# Autodesk Inventor assembly: x_iddler
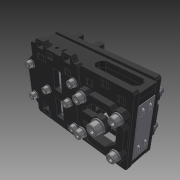
[picture p0: Inventor's stored thumbnail of the model, 180x180]
Saved by Autodesk Inventor 2014 (Build 180170000, 170)
## iProperties
Created: 2014-03-20
Part Number: x_iddler
Document SubType Name: Assembly
Designer: buben
Author: buben
## Documents named in this file (22)
- C:\Users\buben\Documents\GitHub\bacon\inventor files\printer parts\6.5 mm\x_iddler.iam
- C:\Users\buben\Documents\GitHub\bacon\inventor files\printer parts\6.5 mm\x_iddler_bottom.ipt
- C:\Users\buben\Documents\GitHub\bacon\inventor files\printer parts\6.5 mm\x_iddler_belt_bearing_mount.ipt
- C:\Users\buben\Documents\GitHub\bacon\inventor files\printer parts\6.5 mm\x_motor_smooth_rod_spacer.ipt
- C:\Users\buben\Documents\GitHub\bacon\inventor files\printer parts\6.5 mm\x_iddler_wall_lower.ipt
- C:\Users\buben\Documents\GitHub\bacon\inventor files\printer parts\6.5 mm\x_iddler_wall_upper.ipt
- C:\Users\buben\Documents\GitHub\bacon\inventor files\printer parts\6.5 mm\x_iddler_upper_nut_stop.ipt
- C:\Users\buben\Documents\GitHub\bacon\inventor files\printer parts\6.5 mm\x_motor_middle.ipt
- C:\Users\buben\Documents\GitHub\bacon\inventor files\printer parts\6.5 mm\x_iddler_c_mount.ipt
- C:\Users\buben\Documents\GitHub\bacon\inventor files\printer parts\6.5 mm\x_motor_top.ipt
- C:\Users\buben\Documents\GitHub\bacon\inventor files\printer parts\6.5 mm\x_iddler_right_cap.ipt
- C:\Users\buben\Documents\GitHub\bacon\inventor files\utils\washer_m5.ipt
- C:\Users\buben\Documents\GitHub\bacon\inventor files\utils\washer_m6.ipt
- C:\Users\buben\Documents\Inventor\Content Center Files\R2014\en-US\ISO 4762(2)\ISO 4762 - M6 x 60ISO.ipt
- C:\Users\buben\Documents\GitHub\bacon\inventor files\utils\washer_m8.ipt
- C:\Users\buben\Documents\Inventor\Content Center Files\R2014\en-US\ISO 4762(2)\ISO 4762 - M8 x 65ISO.ipt
- C:\Users\buben\Documents\Inventor\Content Center Files\R2014\en-US\ISO 7040\ISO 7040 - M5.ipt
- C:\Users\buben\Documents\Inventor\Content Center Files\R2014\en-US\ISO 7040\ISO 7040 - M6.ipt
- C:\Users\buben\Documents\Inventor\Content Center Files\R2014\en-US\ISO 7040\ISO 7040 - M8.ipt
- C:\Users\buben\Documents\GitHub\bacon\inventor files\3rd party components\linear_bearing_8\Imported Components\LU8MM\LU8MM.iam
- C:\Users\buben\Documents\Inventor\Content Center Files\R2014\en-US\ISO 4762(2)\ISO 4762 - M5 x 50ISO.ipt
- C:\Users\buben\Documents\GitHub\bacon\inventor files\utils\x_iddler_cap_zip_tie.ipt
## Components (62 placed, 21 different names)
1. x_iddler_bottom:1 — Mate:1, Mate:2, Mate:3, Mate:4, Mate:5, Mate:6, Mate:7, Mate:8, Mate:9, Mate:10, Mate:11, Mate:12, Mate:13, Mate:14, Mate:15, Mate:16, Mate:17, Mate:18, Mate:19, Mate:21, Mate:33, Tangent:1, Mate:41, Mate:42, Mate:43, Mate:44, Mate:45, Mate:46
2. x_iddler_belt_bearing_mount:1 — Mate:4, Mate:5, Mate:6, Mate:67, Mate:68, Mate:69, Mate:70, Mate:76, Mate:77
3. x_motor_smooth_rod_spacer:1 — Mate:7, Mate:10, Mate:12, Mate:22
4. x_motor_smooth_rod_spacer:2 — Mate:8, Mate:9, Mate:11
5. x_iddler_wall_lower:1 — Mate:13, Mate:14, Mate:15, Mate:23, Mate:24, Mate:25, Mate:26, Mate:27, Mate:32, Mate:34
6. x_iddler_wall_upper:1 — Mate:16, Mate:17, Mate:18, Mate:20, Mate:31
7. x_iddler_upper_nut_stop:1 — Mate:19, Mate:20, Mate:21
8. x_motor_middle:1 — Mate:22, Mate:23, Mate:24, Mate:101, Mate:102, Mate:103, Mate:104, Mate:106, Mate:107
9. x_iddler_c_mount:1 — Mate:25, Mate:26, Mate:27, Mate:28, Mate:29, Mate:30
10. x_iddler_belt_bearing_mount:2 — Mate:28, Mate:29, Mate:30, Mate:59, Mate:60, Mate:61, Mate:62, Mate:63, Mate:64, Mate:65, Mate:66, Mate:75, Mate:78
11. x_motor_top:1 — Mate:31, Mate:32, Mate:35, Mate:36, Mate:37, Mate:38, Mate:39, Mate:40, Mate:47, Mate:48, Mate:49, Mate:50, Mate:51, Mate:52, Mate:105
12. x_iddler_right_cap:1 — Mate:33, Mate:34, Tangent:1, Angle:1, Angle:2, Angle:3, Angle:4, Tangent:2, Tangent:3, Tangent:4, Tangent:5
13. CSN 02 1702 B B 5,3:1 — Mate:37, Mate:47, Insert:3
14. CSN 02 1702 B B 5,3:2 — Mate:35, Mate:48, Insert:1
15. CSN 02 1702 B B 5,3:3 — Mate:36, Mate:49, Insert:2
16. CSN 02 1702 B B 5,3:4 — Mate:39, Mate:51, Insert:4
17. CSN 02 1702 B B 5,3:5 — Mate:40, Mate:52, Insert:6
18. CSN 02 1702 B B 5,3:6 — Mate:38, Mate:50, Insert:5
19. CSN 02 1702 B B 5,3:7 — Mate:42, Mate:57, Mate:83
20. CSN 02 1702 B B 5,3:8 — Mate:45, Mate:54, Mate:80
21. CSN 02 1702 B B 5,3:9 — Mate:44, Mate:55, Mate:81
22. CSN 02 1702 B B 5,3:10 — Mate:41, Mate:58, Mate:84
23. CSN 02 1702 B B 5,3:11 — Mate:46, Mate:53, Mate:79
24. CSN 02 1702 B B 5,3:12 — Mate:43, Mate:56, Mate:82
25. ISO 4762 M5 x 50:4 — Insert:4, Mate:57, Mate:88
26. ISO 4762 M5 x 50:2 — Insert:3, Mate:54, Mate:85
27. ISO 4762 M5 x 50:1 — Insert:1, Mate:53, Mate:86
28. ISO 4762 M5 x 50:3 — Insert:2, Mate:55, Mate:87
29. ISO 4762 M5 x 50:5 — Insert:6, Mate:58, Mate:89
30. ISO 4762 M5 x 50:6 — Insert:5, Mate:56, Mate:90
31. ISO 4762 M6 x 60:1 — Insert:8, Mate:73, Mate:96
32. ISO 4762 M6 x 60:4 — Insert:9, Mate:71, Mate:98, Mate:108, Mate:109
33. ISO 4762 M6 x 60:2 — Insert:10, Mate:72, Mate:95, Mate:110, Mate:111
34. ISO 4762 M6 x 60:3 — Insert:7, Mate:74, Mate:97
35. CSN 02 1702 B B 6,4:1 — Mate:59, Mate:65, Insert:7
36. CSN 02 1702 B B 6,4:2 — Mate:61, Mate:66, Insert:9
37. CSN 02 1702 B B 6,4:3 — Mate:60, Mate:64, Insert:8
38. CSN 02 1702 B B 6,4:4 — Mate:62, Mate:63, Insert:10
39. CSN 02 1702 B B 6,4:5 — Mate:68, Mate:72, Mate:92
40. CSN 02 1702 B B 6,4:6 — Mate:67, Mate:71, Mate:91
41. CSN 02 1702 B B 6,4:7 — Mate:69, Mate:73, Mate:94
42. CSN 02 1702 B B 6,4:8 — Mate:70, Mate:74, Mate:93
43. CSN 02 1702 B B 8,4:1 — Mate:76, Mate:77, Mate:99
44. CSN 02 1702 B B 8,4:2 — Mate:75, Mate:78, Insert:11
45. ISO 4762 M8 x 65:1 — Insert:11, Mate:100
46. DIN EN ISO 7040 M5:1 — Mate:83, Mate:88
47. DIN EN ISO 7040 M5:2 — Mate:84, Mate:89
48. DIN EN ISO 7040 M5:3 — Mate:80, Mate:85
49. DIN EN ISO 7040 M5:4 — Mate:81, Mate:87
50. DIN EN ISO 7040 M5:5 — Mate:82, Mate:90
51. DIN EN ISO 7040 M5:6 — Mate:79, Mate:86
52. DIN EN ISO 7040 M6:1 — Mate:92, Mate:95
53. DIN EN ISO 7040 M6:2 — Mate:91, Mate:98
54. DIN EN ISO 7040 M6:3 — Mate:94, Mate:96
55. DIN EN ISO 7040 M6:4 — Mate:93, Mate:97
56. DIN EN ISO 7040 M8:1 — Mate:99, Mate:100
57. LU8MM:1 [sub-assembly] — Mate:101, Mate:102, Mate:107
58. LU8MM:2 [sub-assembly] — Mate:103, Mate:104, Mate:105, Mate:106
59. x_iddler_cap_zip_tie:1 — Mate:109, Angle:3, Tangent:3
60. x_iddler_cap_zip_tie:2 — Mate:108, Angle:4, Tangent:5
61. x_iddler_cap_zip_tie:3 — Mate:110, Angle:2, Tangent:2
62. x_iddler_cap_zip_tie:4 — Mate:111, Angle:1, Tangent:4
## Relationships (131: Mate 111, Insert 11, Tangent 5, Angle 4)
- Mate:1: x_iddler_bottom:1
- Mate:2: x_iddler_bottom:1
- Mate:3: x_iddler_bottom:1
- Mate:4: x_iddler_bottom:1 ↔ x_iddler_belt_bearing_mount:1
- Mate:5: x_iddler_bottom:1 ↔ x_iddler_belt_bearing_mount:1
- Mate:6: x_iddler_bottom:1 ↔ x_iddler_belt_bearing_mount:1
- Mate:7: x_iddler_bottom:1 ↔ x_motor_smooth_rod_spacer:1
- Mate:8: x_iddler_bottom:1 ↔ x_motor_smooth_rod_spacer:2
- Mate:9: x_iddler_bottom:1 ↔ x_motor_smooth_rod_spacer:2
- Mate:10: x_iddler_bottom:1 ↔ x_motor_smooth_rod_spacer:1
- Mate:11: x_iddler_bottom:1 ↔ x_motor_smooth_rod_spacer:2
- Mate:12: x_iddler_bottom:1 ↔ x_motor_smooth_rod_spacer:1
- Mate:13: x_iddler_bottom:1 ↔ x_iddler_wall_lower:1
- Mate:14: x_iddler_bottom:1 ↔ x_iddler_wall_lower:1
- Mate:15: x_iddler_bottom:1 ↔ x_iddler_wall_lower:1
- Mate:16: x_iddler_bottom:1 ↔ x_iddler_wall_upper:1
- Mate:17: x_iddler_bottom:1 ↔ x_iddler_wall_upper:1
- Mate:18: x_iddler_bottom:1 ↔ x_iddler_wall_upper:1
- Mate:19: x_iddler_bottom:1 ↔ x_iddler_upper_nut_stop:1
- Mate:20: x_iddler_wall_upper:1 ↔ x_iddler_upper_nut_stop:1
- Mate:21: x_iddler_bottom:1 ↔ x_iddler_upper_nut_stop:1
- Mate:22: x_motor_smooth_rod_spacer:1 ↔ x_motor_middle:1
- Mate:23: x_iddler_wall_lower:1 ↔ x_motor_middle:1
- Mate:24: x_iddler_wall_lower:1 ↔ x_motor_middle:1
- Mate:25: x_iddler_wall_lower:1 ↔ x_iddler_c_mount:1
- Mate:26: x_iddler_wall_lower:1 ↔ x_iddler_c_mount:1
- Mate:27: x_iddler_wall_lower:1 ↔ x_iddler_c_mount:1
- Mate:28: x_iddler_c_mount:1 ↔ x_iddler_belt_bearing_mount:2
- Mate:29: x_iddler_c_mount:1 ↔ x_iddler_belt_bearing_mount:2
- Mate:30: x_iddler_c_mount:1 ↔ x_iddler_belt_bearing_mount:2
- Mate:31: x_iddler_wall_upper:1 ↔ x_motor_top:1
- Mate:32: x_iddler_wall_lower:1 ↔ x_motor_top:1
- Mate:33: x_iddler_bottom:1 ↔ x_iddler_right_cap:1
- Mate:34: x_iddler_wall_lower:1 ↔ x_iddler_right_cap:1
- Tangent:1: x_iddler_bottom:1 ↔ x_iddler_right_cap:1
- Mate:35: x_motor_top:1 ↔ CSN 02 1702 B B 5,3:2
- Mate:36: x_motor_top:1 ↔ CSN 02 1702 B B 5,3:3
- Mate:37: x_motor_top:1 ↔ CSN 02 1702 B B 5,3:1
- Mate:38: x_motor_top:1 ↔ CSN 02 1702 B B 5,3:6
- Mate:39: x_motor_top:1 ↔ CSN 02 1702 B B 5,3:4
- Mate:40: x_motor_top:1 ↔ CSN 02 1702 B B 5,3:5
- Mate:41: x_iddler_bottom:1 ↔ CSN 02 1702 B B 5,3:10
- Mate:42: x_iddler_bottom:1 ↔ CSN 02 1702 B B 5,3:7
- Mate:43: x_iddler_bottom:1 ↔ CSN 02 1702 B B 5,3:12
- Mate:44: x_iddler_bottom:1 ↔ CSN 02 1702 B B 5,3:9
- Mate:45: x_iddler_bottom:1 ↔ CSN 02 1702 B B 5,3:8
- Mate:46: x_iddler_bottom:1 ↔ CSN 02 1702 B B 5,3:11
- Mate:47: x_motor_top:1 ↔ CSN 02 1702 B B 5,3:1
- Mate:48: x_motor_top:1 ↔ CSN 02 1702 B B 5,3:2
- Mate:49: x_motor_top:1 ↔ CSN 02 1702 B B 5,3:3
- Mate:50: x_motor_top:1 ↔ CSN 02 1702 B B 5,3:6
- Mate:51: x_motor_top:1 ↔ CSN 02 1702 B B 5,3:4
- Mate:52: x_motor_top:1 ↔ CSN 02 1702 B B 5,3:5
- Insert:1: CSN 02 1702 B B 5,3:2 ↔ ISO 4762 M5 x 50:1
- Insert:2: CSN 02 1702 B B 5,3:3 ↔ ISO 4762 M5 x 50:3
- Insert:3: CSN 02 1702 B B 5,3:1 ↔ ISO 4762 M5 x 50:2
- Insert:4: CSN 02 1702 B B 5,3:4 ↔ ISO 4762 M5 x 50:4
- Insert:5: CSN 02 1702 B B 5,3:6 ↔ ISO 4762 M5 x 50:6
- Insert:6: CSN 02 1702 B B 5,3:5 ↔ ISO 4762 M5 x 50:5
- Mate:53: CSN 02 1702 B B 5,3:11 ↔ ISO 4762 M5 x 50:1
- Mate:54: CSN 02 1702 B B 5,3:8 ↔ ISO 4762 M5 x 50:2
- Mate:55: CSN 02 1702 B B 5,3:9 ↔ ISO 4762 M5 x 50:3
- Mate:56: CSN 02 1702 B B 5,3:12 ↔ ISO 4762 M5 x 50:6
- Mate:57: CSN 02 1702 B B 5,3:7 ↔ ISO 4762 M5 x 50:4
- Mate:58: CSN 02 1702 B B 5,3:10 ↔ ISO 4762 M5 x 50:5
- Mate:59: x_iddler_belt_bearing_mount:2 ↔ CSN 02 1702 B B 6,4:1
- Mate:60: x_iddler_belt_bearing_mount:2 ↔ CSN 02 1702 B B 6,4:3
- Mate:61: x_iddler_belt_bearing_mount:2 ↔ CSN 02 1702 B B 6,4:2
- Mate:62: x_iddler_belt_bearing_mount:2 ↔ CSN 02 1702 B B 6,4:4
- Mate:63: x_iddler_belt_bearing_mount:2 ↔ CSN 02 1702 B B 6,4:4
- Mate:64: x_iddler_belt_bearing_mount:2 ↔ CSN 02 1702 B B 6,4:3
- Mate:65: x_iddler_belt_bearing_mount:2 ↔ CSN 02 1702 B B 6,4:1
- Mate:66: x_iddler_belt_bearing_mount:2 ↔ CSN 02 1702 B B 6,4:2
- Insert:7: ISO 4762 M6 x 60:3 ↔ CSN 02 1702 B B 6,4:1
- Insert:8: ISO 4762 M6 x 60:1 ↔ CSN 02 1702 B B 6,4:3
- Insert:9: ISO 4762 M6 x 60:4 ↔ CSN 02 1702 B B 6,4:2
- Insert:10: ISO 4762 M6 x 60:2 ↔ CSN 02 1702 B B 6,4:4
- Mate:67: x_iddler_belt_bearing_mount:1 ↔ CSN 02 1702 B B 6,4:6
- Mate:68: x_iddler_belt_bearing_mount:1 ↔ CSN 02 1702 B B 6,4:5
- Mate:69: x_iddler_belt_bearing_mount:1 ↔ CSN 02 1702 B B 6,4:7
- Mate:70: x_iddler_belt_bearing_mount:1 ↔ CSN 02 1702 B B 6,4:8
- Mate:71: ISO 4762 M6 x 60:4 ↔ CSN 02 1702 B B 6,4:6
- Mate:72: ISO 4762 M6 x 60:2 ↔ CSN 02 1702 B B 6,4:5
- Mate:73: ISO 4762 M6 x 60:1 ↔ CSN 02 1702 B B 6,4:7
- Mate:74: ISO 4762 M6 x 60:3 ↔ CSN 02 1702 B B 6,4:8
- Mate:75: x_iddler_belt_bearing_mount:2 ↔ CSN 02 1702 B B 8,4:2
- Mate:76: x_iddler_belt_bearing_mount:1 ↔ CSN 02 1702 B B 8,4:1
- Mate:77: x_iddler_belt_bearing_mount:1 ↔ CSN 02 1702 B B 8,4:1
- Mate:78: x_iddler_belt_bearing_mount:2 ↔ CSN 02 1702 B B 8,4:2
- Insert:11: CSN 02 1702 B B 8,4:2 ↔ ISO 4762 M8 x 65:1
- Mate:79: CSN 02 1702 B B 5,3:11 ↔ DIN EN ISO 7040 M5:6
- Mate:80: CSN 02 1702 B B 5,3:8 ↔ DIN EN ISO 7040 M5:3
- Mate:81: CSN 02 1702 B B 5,3:9 ↔ DIN EN ISO 7040 M5:4
- Mate:82: CSN 02 1702 B B 5,3:12 ↔ DIN EN ISO 7040 M5:5
- Mate:83: CSN 02 1702 B B 5,3:7 ↔ DIN EN ISO 7040 M5:1
- Mate:84: CSN 02 1702 B B 5,3:10 ↔ DIN EN ISO 7040 M5:2
- Mate:85: ISO 4762 M5 x 50:2 ↔ DIN EN ISO 7040 M5:3
- Mate:86: ISO 4762 M5 x 50:1 ↔ DIN EN ISO 7040 M5:6
- Mate:87: ISO 4762 M5 x 50:3 ↔ DIN EN ISO 7040 M5:4
- Mate:88: ISO 4762 M5 x 50:4 ↔ DIN EN ISO 7040 M5:1
- Mate:89: ISO 4762 M5 x 50:5 ↔ DIN EN ISO 7040 M5:2
- Mate:90: ISO 4762 M5 x 50:6 ↔ DIN EN ISO 7040 M5:5
- Mate:91: CSN 02 1702 B B 6,4:6 ↔ DIN EN ISO 7040 M6:2
- Mate:92: CSN 02 1702 B B 6,4:5 ↔ DIN EN ISO 7040 M6:1
- Mate:93: CSN 02 1702 B B 6,4:8 ↔ DIN EN ISO 7040 M6:4
- Mate:94: CSN 02 1702 B B 6,4:7 ↔ DIN EN ISO 7040 M6:3
- Mate:95: ISO 4762 M6 x 60:2 ↔ DIN EN ISO 7040 M6:1
- Mate:96: ISO 4762 M6 x 60:1 ↔ DIN EN ISO 7040 M6:3
- Mate:97: ISO 4762 M6 x 60:3 ↔ DIN EN ISO 7040 M6:4
- Mate:98: ISO 4762 M6 x 60:4 ↔ DIN EN ISO 7040 M6:2
- Mate:99: CSN 02 1702 B B 8,4:1 ↔ DIN EN ISO 7040 M8:1
- Mate:100: ISO 4762 M8 x 65:1 ↔ DIN EN ISO 7040 M8:1
- Mate:101 (7.5 mm): x_motor_middle:1 ↔ LU8MM:1
- Mate:102 (7.5 mm): x_motor_middle:1 ↔ LU8MM:1
- Mate:103 (7.5 mm): x_motor_middle:1 ↔ LU8MM:2
- Mate:104 (7.5 mm): x_motor_middle:1 ↔ LU8MM:2
- Mate:105 (7.5 mm): x_motor_top:1 ↔ LU8MM:2
- Mate:106 (0.5 mm): x_motor_middle:1 ↔ LU8MM:2
- Mate:107 (0.5 mm): x_motor_middle:1 ↔ LU8MM:1
- Mate:108: ISO 4762 M6 x 60:4 ↔ x_iddler_cap_zip_tie:2
- Mate:109: ISO 4762 M6 x 60:4 ↔ x_iddler_cap_zip_tie:1
- Mate:110: ISO 4762 M6 x 60:2 ↔ x_iddler_cap_zip_tie:3
- Mate:111: ISO 4762 M6 x 60:2 ↔ x_iddler_cap_zip_tie:4
- Angle:1 (180 deg): x_iddler_right_cap:1 ↔ x_iddler_cap_zip_tie:4
- Angle:2 (180 deg): x_iddler_right_cap:1 ↔ x_iddler_cap_zip_tie:3
- Angle:3 (180 deg): x_iddler_right_cap:1 ↔ x_iddler_cap_zip_tie:1
- Angle:4 (180 deg): x_iddler_right_cap:1 ↔ x_iddler_cap_zip_tie:2
- Tangent:2: x_iddler_right_cap:1 ↔ x_iddler_cap_zip_tie:3
- Tangent:3: x_iddler_right_cap:1 ↔ x_iddler_cap_zip_tie:1
- Tangent:4: x_iddler_right_cap:1 ↔ x_iddler_cap_zip_tie:4
- Tangent:5: x_iddler_right_cap:1 ↔ x_iddler_cap_zip_tie:2
